# Autodesk Inventor assembly: UjKertIstaloElott
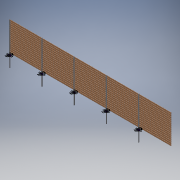
[picture p0: Inventor's stored thumbnail of the model, 180x180]
Saved by Autodesk Inventor 2019 (Build 230136000, 136)
## iProperties
Created: 2025-01-08
Part Number: UjKertIstaloElott
Document SubType Name: Assembly
Designer: laca
Author: laca
## Documents named in this file (2)
- C:\Users\laca\Documents\Inventor\Kerites\UjKertIstaloElott.iam
- C:\Users\laca\Documents\Inventor\Kerites\1LabKert.iam
## Components (5 placed, 1 different names)
1. 1LabKert:1 [sub-assembly]
2. 1LabKert:2 [sub-assembly]
3. 1LabKert:3 [sub-assembly]
4. 1LabKert:4 [sub-assembly]
5. 1LabKert:5 [sub-assembly]
## Component patterns: (5 elements, first: 1LabKert:1)
